# Autodesk Inventor assembly: bellows_latest
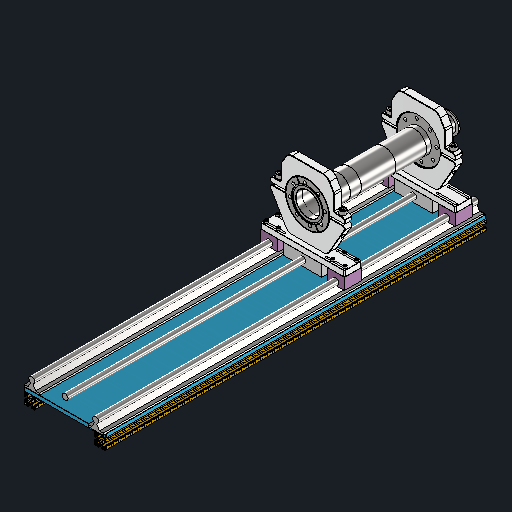
[picture p0: Inventor's stored thumbnail of the model, 512x512]
Saved by Autodesk Inventor 2027.1 (Build 311270010, 270A)
## iProperties
Created: 2026-06-04
Part Number: bellows_latest
Document SubType Name: Assembly
Designer: shusu
Author: shusu
## Documents named in this file (12)
- C:\Users\queezz\Dropbox\Drawings\pihti-cad\bellows-probe\sliding-assembly.iam
- C:\Users\queezz\Dropbox\Drawings\pihti-cad\bellows-probe\rail bwllows probe.ipt
- C:\Users\queezz\Dropbox\Drawings\pihti-cad\bellows-probe\Al-profile-30x30-L1000.ipt
- C:\Users\queezz\Dropbox\Drawings\pihti-cad\ContentCenter\Aluminium-profiles\Al-profile-30x30.ipt
- C:\Users\queezz\Dropbox\Drawings\pihti-cad\bellows-probe\base-plate-for-bellows.ipt
- C:\Users\queezz\Dropbox\Drawings\pihti-cad\ContentCenter\Fastners\M6x16-SHCS.ipt
- C:\Users\queezz\Dropbox\Drawings\pihti-cad\ContentCenter\Fastners\M5x20-SHCS.ipt
- C:\Users\queezz\Dropbox\Drawings\pihti-cad\ContentCenter\CF-KF-adapters\ICF70_to_KF40.ipt
- C:\Users\queezz\Dropbox\Drawings\pihti-cad\bellows-probe\CF114-CF70-zero-length-adappter.ipt
- C:\Users\queezz\Dropbox\Drawings\pihti-cad\bellows-probe\M16-lead-screw.ipt
- C:\Users\queezz\Dropbox\Drawings\pihti-cad\bellows-probe\lead-screw-nut-preview.ipt
- C:\Users\queezz\Dropbox\Drawings\pihti-cad\bellows-probe\bellows-clamped-on-bearings.iam
## Components (20 placed, 10 different names)
1. rail:1 — Mate:9
2. rail:2 — Mate:9, Mate:16, Flush:12, Flush:20
3. Al-profile-30x30-L1000:1 — Mate:18, Flush:13, Flush:16
4. Al-profile-30x30-L1000:2 — Mate:17, Flush:14, Flush:15
5. base-plate-for-bellows:1 — Mate:16, Flush:11, Flush:12, Mate:17, Mate:18, Flush:13, Flush:14, Flush:15, Flush:16
6. ICF70_to_KF40:1 — Rotational:6
7. CF114-CF70-zero-length-adappter:1 — Rotational:6
8. M16-lead-screw:1 — Mate:26, Flush:20
9. lead-screw-nut-preview:1 — Mate:26
10. lead-screw-nut-preview:2
11. bellows-clamped-on-bearings:1 [sub-assembly]
12. JIS B 1176 - Metric M6 x 16:2
13. JIS B 1176 - Metric M6 x 16:3
14. JIS B 1176 - Metric M6 x 16:4
15. AS 1420 - Metric M5 x 20:1
16. AS 1420 - Metric M5 x 20:2
17. AS 1420 - Metric M5 x 20:3
18. AS 1420 - Metric M5 x 20:4
19. AS 1420 - Metric M5 x 20:7
20. JIS B 1176 - Metric M6 x 16:1
## Relationships (31: Mate 11, WeldJoint 8, Flush 7, RevoluteJoint 5)
- [Mate]: rail:1 ↔ bellows-clamped-on-bearings:1
- [Mate]: rail:2 ↔ bellows-clamped-on-bearings:1
- [Mate]: rail:2 ↔ bellows-clamped-on-bearings:1
- [Mate]: rail:1 ↔ bellows-clamped-on-bearings:1
- Mate:9 (175 mm): rail:1 ↔ rail:2
- [Mate]: bellows-clamped-on-bearings:1
- [Mate]: bellows-clamped-on-bearings:1
- Mate:16: rail:2 ↔ base-plate-for-bellows:1
- Flush:11: base-plate-for-bellows:1
- Flush:12: rail:2 ↔ base-plate-for-bellows:1
- Mate:17: Al-profile-30x30-L1000:2 ↔ base-plate-for-bellows:1
- Mate:18: Al-profile-30x30-L1000:1 ↔ base-plate-for-bellows:1
- Flush:13: Al-profile-30x30-L1000:1 ↔ base-plate-for-bellows:1
- Flush:14: Al-profile-30x30-L1000:2 ↔ base-plate-for-bellows:1
- Flush:15: Al-profile-30x30-L1000:2 ↔ base-plate-for-bellows:1
- Flush:16: Al-profile-30x30-L1000:1 ↔ base-plate-for-bellows:1
- [WeldJoint]: bellows-clamped-on-bearings:1 ↔ JIS B 1176 - Metric M6 x 16:1
- [WeldJoint]: bellows-clamped-on-bearings:1 ↔ JIS B 1176 - Metric M6 x 16:2
- [WeldJoint]: bellows-clamped-on-bearings:1 ↔ JIS B 1176 - Metric M6 x 16:3
- [WeldJoint]: bellows-clamped-on-bearings:1 ↔ JIS B 1176 - Metric M6 x 16:4
- [RevoluteJoint] (15 mm): bellows-clamped-on-bearings:1 ↔ AS 1420 - Metric M5 x 20:1
- [RevoluteJoint] (15 mm): bellows-clamped-on-bearings:1 ↔ AS 1420 - Metric M5 x 20:3
- [RevoluteJoint] (15 mm): bellows-clamped-on-bearings:1 ↔ AS 1420 - Metric M5 x 20:2
- [RevoluteJoint] (15 mm): bellows-clamped-on-bearings:1 ↔ AS 1420 - Metric M5 x 20:7
- [WeldJoint] (15 mm): bellows-clamped-on-bearings:1 ↔ AS 1420 - Metric M5 x 20:4
- [WeldJoint]: CF114-CF70-zero-length-adappter:1 ↔ bellows-clamped-on-bearings:1
- Rotational:6 [RevoluteJoint]: ICF70_to_KF40:1 ↔ CF114-CF70-zero-length-adappter:1
- Mate:26: M16-lead-screw:1 ↔ lead-screw-nut-preview:1
- Flush:20: rail:2 ↔ M16-lead-screw:1
- [WeldJoint]: lead-screw-nut-preview:1 ↔ bellows-clamped-on-bearings:1
- [WeldJoint]: lead-screw-nut-preview:2 ↔ bellows-clamped-on-bearings:1
